# Autodesk Inventor assembly: Shelf Holder Joint11
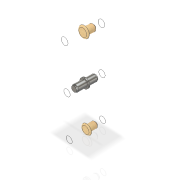
[picture p0: Inventor's stored thumbnail of the model, 180x180]
Saved by Autodesk Inventor 2024 (Build 280153000, 153)
## iProperties
RuleStatus: InUse
Created: 2023-02-06
Part Number: Shelf Holder Joint11
Document SubType Name: Assembly
Designer: sauliusd
Author: sauliusd
## Documents named in this file (4)
- C:\W4INV 2024 Design\PROJECTS\Samples\Macro DEMO\7 Computer Case\Computer Case.iam Smart Hardware\Shelf Holder Joint11\Shelf Holder Joint11.iam
- C:\W4INV 2024 Design\PROJECTS\Samples\Macro DEMO\7 Computer Case\Computer Case.iam Smart Hardware\Shelf Holder Joint11\Shelf Holder Joint1100.ipt
- C:\W4INV 2022 Design\LIBRARY\Holders\Shelf holder D5.ipt
- C:\W4INV 2024 Design\_LIBRARY\Holders\Shelf holder D5\Shelf support D5 L16 with hole covers.ipt
## Components (3 placed, 3 different names)
1. @Skeleton — Flush:1, Flush:2, Flush:3, Insert:1
2. Shelf Support D5 — Insert:1, Angle:1
3. Shelf support D5 L16 with hole covers:2
## Component patterns: (2 elements, first: Shelf Support D5)
## Relationships (5: Flush 3, Insert 1, Angle 1)
- Flush:1: @Skeleton
- Flush:2: @Skeleton
- Flush:3: @Skeleton
- Insert:1: @Skeleton ↔ Shelf Support D5
- Angle:1 (0 deg): Shelf Support D5
## Named parameters: ContactPatchHeight = 18 mm, ContactPatchWidth = 583 mm, PillarBoardT = 18 mm, HoleNumber = 3
